# Autodesk Inventor assembly: Assembly1
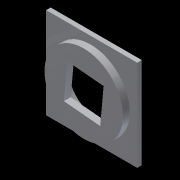
[picture p0: Inventor's stored thumbnail of the model, 180x180]
Saved by Autodesk Inventor 2014 SP1 (Build 180222100, 222)
## iProperties
Created: 2014-04-13
Part Number: Assembly1
Document SubType Name: Assembly
Designer: Rauhul Varma
Mass: 133.546 g
Surface Area: 498.694 cm^2
Volume: 133.643 cm^3
Density: 0.999278 g/cm^3
Author: Rauhul Varma
## Documents named in this file (4)
- C:\Users\Rauhul Varma\Desktop\Low CoG Swerve\Assembly1.iam
- C:\Users\Rauhul Varma\Desktop\Low CoG Swerve\Upper Plate.ipt
- C:\Users\Rauhul Varma\Desktop\Low CoG Swerve\Ball.ipt
- C:\Users\Rauhul Varma\Desktop\Low CoG Swerve\Base Gear.ipt
## Components (17 placed, 3 different names)
1. Upper Plate:1 — Mate:1, Tangent:1, Tangent:3, Tangent:4, Tangent:5, Tangent:6, Tangent:7, Tangent:8, Tangent:9, Tangent:10, Tangent:11, Tangent:12, Tangent:13, Tangent:14, Tangent:15, Tangent:16
2. Ball:1 — Tangent:1, Tangent:2, Tangent:19, Tangent:20
3. Base Gear:1 — Mate:1, Tangent:2
4. Ball:2 — Tangent:16, Tangent:17
5. Ball:3 — Tangent:8
6. Ball:4 — Tangent:3, Tangent:22, Tangent:23
7. Ball:5 — Tangent:4
8. Ball:6 — Tangent:11
9. Ball:7 — Tangent:5, Tangent:25
10. Ball:8 — Tangent:14, Tangent:24, Tangent:25
11. Ball:9 — Tangent:12, Tangent:17, Tangent:18
12. Ball:10 — Tangent:15, Tangent:20, Tangent:21
13. Ball:11 — Tangent:13
14. Ball:12 — Tangent:10, Tangent:23, Tangent:24
15. Ball:13 — Tangent:9, Tangent:21, Tangent:22
16. Ball:14 — Tangent:7
17. Ball:15 — Tangent:6, Tangent:18, Tangent:19
## Relationships (26: Tangent 25, Mate 1)
- Mate:1: Upper Plate:1 ↔ Base Gear:1
- Tangent:1: Upper Plate:1 ↔ Ball:1
- Tangent:2: Ball:1 ↔ Base Gear:1
- Tangent:3: Upper Plate:1 ↔ Ball:4
- Tangent:4: Upper Plate:1 ↔ Ball:5
- Tangent:5: Upper Plate:1 ↔ Ball:7
- Tangent:6: Upper Plate:1 ↔ Ball:15
- Tangent:7: Upper Plate:1 ↔ Ball:14
- Tangent:8: Upper Plate:1 ↔ Ball:3
- Tangent:9: Upper Plate:1 ↔ Ball:13
- Tangent:10: Upper Plate:1 ↔ Ball:12
- Tangent:11: Upper Plate:1 ↔ Ball:6
- Tangent:12: Upper Plate:1 ↔ Ball:9
- Tangent:13: Upper Plate:1 ↔ Ball:11
- Tangent:14: Upper Plate:1 ↔ Ball:8
- Tangent:15: Upper Plate:1 ↔ Ball:10
- Tangent:16: Upper Plate:1 ↔ Ball:2
- Tangent:17 (0.1016 mm): Ball:2 ↔ Ball:9
- Tangent:18 (0.1016 mm): Ball:9 ↔ Ball:15
- Tangent:19 (0.1016 mm): Ball:1 ↔ Ball:15
- Tangent:20 (0.1016 mm): Ball:1 ↔ Ball:10
- Tangent:21 (0.1016 mm): Ball:10 ↔ Ball:13
- Tangent:22 (0.1016 mm): Ball:4 ↔ Ball:13
- Tangent:23 (0.1016 mm): Ball:4 ↔ Ball:12
- Tangent:24 (0.1016 mm): Ball:8 ↔ Ball:12
- Tangent:25 (0.1016 mm): Ball:7 ↔ Ball:8
